# Autodesk Inventor assembly: HD-Motor-Mount
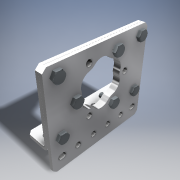
[picture p0: Inventor's stored thumbnail of the model, 180x180]
Saved by Autodesk Inventor 2017.3 (Build 213256000, 256)
## iProperties
Created: 2018-01-05
Part Number: HD-Motor-Mount
Document SubType Name: Assembly
Designer: pranav
Author: pranav
## iProperties of the stored document REV-41-1027A.ipt
Created: 2016-11-16
Part Number: REV-41-1027A
Material: Generic
Description: STEP AP214
Document SubType Name: Modeling
Designer: pranav
Density: 1 g/cm^3
Appearance: Default
Sending System: SolidWorks 2015
Preprocessor: SwSTEP 2.0
Title: REV-41-1027A.STEP
Revision Number: ANY
## iProperties of the stored document REV-41-1027B.ipt
Created: 2015-08-20
Part Number: REV-41-1027B
Material: Generic
Description: STEP AP214
Document SubType Name: Modeling
Designer: pranav
Density: 1 g/cm^3
Appearance: Default
Sending System: SolidWorks 2014
Preprocessor: SwSTEP 2.0
Title: REV-41-1027.STEP
Revision Number: ANY
## iProperties of the stored document REV-41-1361 Simple.ipt
Created: 2017-04-10
Part Number: REV-41-1361 Simple
Material: Generic
Document SubType Name: Modeling
Designer: pranav
Density: 1 g/cm^3
Appearance: Default
Sending System: Autodesk Translation Framework v5.2.0.2920
Preprocessor: ST-DEVELOPER v16.5
Title: E:/Dropbox/REV Robotics/STEP Files/REV-41-1361 Simple.step
## iProperties of the stored document REV-41-1359 Simple.ipt
Created: 2017-04-10
Part Number: REV-41-1359 Simple
Material: Generic
Document SubType Name: Modeling
Designer: pranav
Density: 1 g/cm^3
Appearance: Default
Sending System: Autodesk Translation Framework v5.2.0.2920
Preprocessor: ST-DEVELOPER v16.5
Title: E:/Dropbox/REV Robotics/STEP Files/REV-41-1359 Simple.step
## Documents named in this file (9)
- **C:\Users\pranav\Documents\Inventor\REV-Robot-CAD\HD-Motor-Mount.iam*LocalDocs*xBkst2s0pBlpeuyo4Vzxv45x50b*REV-41-1027A.ipt
- **C:\Users\pranav\Documents\Inventor\REV-Robot-CAD\HD-Motor-Mount.iam*LocalDocs*x43utpe5fOjqkehwiC0yd1m5dYb*REV-41-1027B.ipt
- **C:\Users\pranav\Documents\Inventor\REV-Robot-CAD\HD-Motor-Mount.iam*LocalDocs*xC0f235bgEatdu1oaMklsyo3bAc*REV-41-1361 Simple.ipt
- **C:\Users\pranav\Documents\Inventor\REV-Robot-CAD\HD-Motor-Mount.iam*LocalDocs*xXtlhfps2Elwfuycb5kdmmt30Sf*REV-41-1359 Simple.ipt
- C:\Users\pranav\Documents\Inventor\REV-Robot-CAD\HD-Motor-Mount.iam
- C:\Users\pranav\Documents\Inventor\REV-Robot-CAD\REV Robotics\REV Robotics CAD\REV-41-1027A.STEP
- C:\Users\pranav\Documents\Inventor\REV-Robot-CAD\REV Robotics\REV Robotics CAD\REV-41-1027B.STEP
- C:\Users\pranav\Documents\Inventor\REV-Robot-CAD\REV Robotics\REV Robotics CAD\REV-41-1359 Simple.step
- C:\Users\pranav\Documents\Inventor\REV-Robot-CAD\REV Robotics\REV Robotics CAD\REV-41-1361 Simple.step
## Components (13 placed, 4 different names)
1. REV-41-1027A:1 — Flush:2, Flush:3, Mate:8, Mate:9, Mate:10, Mate:11
2. REV-41-1027B:1 — Flush:2, Flush:3, Mate:12, Mate:13, Mate:14, Mate:15, Mate:16, Mate:17, Mate:18, Mate:19
3. REV-41-1359 Simple:1 — Mate:8, Mate:12, Mate:22
4. REV-41-1359 Simple:2
5. REV-41-1359 Simple:3
6. REV-41-1359 Simple:4
7. REV-41-1359 Simple:5 — Mate:10, Mate:15, Mate:21
8. REV-41-1359 Simple:6 — Mate:9, Mate:14, Mate:23
9. REV-41-1359 Simple:7 — Mate:11, Mate:13, Mate:20
10. REV-41-1361 Simple:1 — Mate:17, Mate:22
11. REV-41-1361 Simple:2 — Mate:19, Mate:20
12. REV-41-1361 Simple:3 — Mate:18, Mate:21
13. REV-41-1361 Simple:4 — Mate:16, Mate:23
## Relationships (18: Mate 16, Flush 2)
- Flush:2: REV-41-1027A:1 ↔ REV-41-1027B:1
- Flush:3: REV-41-1027A:1 ↔ REV-41-1027B:1
- Mate:8: REV-41-1027A:1 ↔ REV-41-1359 Simple:1
- Mate:9: REV-41-1027A:1 ↔ REV-41-1359 Simple:6
- Mate:10: REV-41-1027A:1 ↔ REV-41-1359 Simple:5
- Mate:11: REV-41-1027A:1 ↔ REV-41-1359 Simple:7
- Mate:12: REV-41-1027B:1 ↔ REV-41-1359 Simple:1
- Mate:13: REV-41-1027B:1 ↔ REV-41-1359 Simple:7
- Mate:14: REV-41-1027B:1 ↔ REV-41-1359 Simple:6
- Mate:15: REV-41-1027B:1 ↔ REV-41-1359 Simple:5
- Mate:16: REV-41-1027B:1 ↔ REV-41-1361 Simple:4
- Mate:17: REV-41-1027B:1 ↔ REV-41-1361 Simple:1
- Mate:18: REV-41-1027B:1 ↔ REV-41-1361 Simple:3
- Mate:19: REV-41-1027B:1 ↔ REV-41-1361 Simple:2
- Mate:20: REV-41-1359 Simple:7 ↔ REV-41-1361 Simple:2
- Mate:21: REV-41-1359 Simple:5 ↔ REV-41-1361 Simple:3
- Mate:22: REV-41-1359 Simple:1 ↔ REV-41-1361 Simple:1
- Mate:23: REV-41-1359 Simple:6 ↔ REV-41-1361 Simple:4
